# Autodesk Inventor assembly: printer
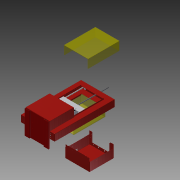
[picture p0: Inventor's stored thumbnail of the model, 180x180]
Saved by Autodesk Inventor 2014 SP2 (Build 180246200, 246)
## iProperties
Created: 2016-09-18
Part Number: printer
Document SubType Name: Assembly
Designer: cruiser
Mass: 5383.42 g
Surface Area: 18310.6 cm^2
Volume: 1570.17 cm^3
Density: 3.42856 g/cm^3
Author: cruiser
## Documents named in this file (18)
- C:\Users\cruiser\Desktop\models\3d printers\laserresin5\printer.iam
- C:\Users\cruiser\Desktop\models\3d printers\laserresin5\frame_front.ipt
- C:\Users\cruiser\Desktop\models\3d printers\laserresin5\frame_back.ipt
- C:\Users\cruiser\Desktop\models\3d printers\laserresin5\drawer.ipt
- C:\Users\cruiser\Desktop\models\3d printers\laserresin5\reservoir.ipt
- C:\Users\cruiser\Desktop\models\3d printers\laserresin5\tray.ipt
- C:\Users\cruiser\Desktop\models\3d printers\laserresin5\crane.ipt
- C:\Users\cruiser\Desktop\models\3d printers\laserresin5\platform.ipt
- C:\Users\cruiser\Desktop\models\3d printers\laserresin5\handle.ipt
- C:\Users\cruiser\Desktop\models\3d printers\laserresin5\laserholder.ipt
- C:\Users\cruiser\Desktop\models\3d printers\laserresin5\nema17.ipt
- C:\Users\cruiser\Desktop\models\3d printers\laserresin5\lmk8luu.ipt
- C:\Users\cruiser\Desktop\models\3d printers\laserresin5\threaded_rod.ipt
- C:\Users\cruiser\Desktop\models\3d printers\laserresin5\shf8.ipt
- C:\Users\cruiser\Desktop\models\3d printers\laserresin5\m8_rail.ipt
- C:\Users\cruiser\Desktop\models\3d printers\laserresin5\foot.ipt
- C:\Users\cruiser\Desktop\models\3d printers\laserresin5\shield.ipt
- C:\Users\cruiser\Desktop\models\3d printers\laserresin5\drawer_pcb.ipt
## Components (24 placed, 17 different names)
1. frame_front:1 — Mate:1, Mate:8, Mate:9, Mate:17, Mate:19, Mate:26, Mate:38, Mate:39, Mate:40, Mate:41, Mate:42, Mate:43, Mate:44, Mate:45, Mate:46, Mate:47, Mate:48, Mate:49, Flush:7, Flush:8, Mate:60, Mate:61, Mate:67
2. frame_back:1 — Mate:60, Mate:61, Mate:64, Mate:65, Mate:66
3. drawer:1 — Mate:1, Mate:19, Mate:23, Mate:24, Mate:26, Mate:54, Mate:57, Mate:58, Mate:59, Mate:62
4. reservoir:1 — Mate:5, Flush:4, Mate:13, Mate:14, Mate:15, Mate:16, Mate:23, Mate:24, Flush:6, Mate:59
5. tray:1 — Mate:5, Flush:4, Flush:6
6. crane:1 — Mate:6, Mate:8, Mate:9, Mate:27, Mate:28, Mate:29, Mate:30, Mate:31, Mate:32, Mate:33, Mate:34, Mate:35, Mate:52, Mate:53
7. platform:1 — Mate:6, Mate:52, Mate:53
8. handle:1 — Mate:13, Mate:14
9. handle:2 — Mate:15, Mate:16
10. laserholder:1 — Mate:17
11. nema17:1 — Mate:27, Mate:28, Mate:29, Mate:36, Mate:37
12. lmk8luu:1 — Mate:30, Mate:34, Mate:35
13. lmk8luu:2 — Mate:31, Mate:32, Mate:33
14. threaded_rod:1 — Mate:36, Mate:37
15. shf8:1 — Mate:44, Mate:45, Mate:46
16. shf8:2 — Mate:41, Mate:42, Mate:43
17. shf8:3 — Mate:47, Mate:48, Mate:49, Mate:51
18. shf8:4 — Mate:38, Mate:39, Mate:40, Mate:50
19. m8_rail:1 — Mate:50, Flush:7
20. m8_rail:2 — Mate:51, Flush:8
21. foot:1 — Mate:54, Mate:57, Mate:58
22. shield:1 — Mate:62
23. shield:2 — Mate:64, Mate:68
24. drawer_pcb:1 — Mate:65, Mate:66, Mate:67, Mate:68
## Relationships (57: Mate 53, Flush 4)
- Mate:1: frame_front:1 ↔ drawer:1
- Mate:5: reservoir:1 ↔ tray:1
- Flush:4: reservoir:1 ↔ tray:1
- Mate:6: crane:1 ↔ platform:1
- Mate:8: frame_front:1 ↔ crane:1
- Mate:9: frame_front:1 ↔ crane:1
- Mate:13: reservoir:1 ↔ handle:1
- Mate:14: reservoir:1 ↔ handle:1
- Mate:15: reservoir:1 ↔ handle:2
- Mate:16: reservoir:1 ↔ handle:2
- Mate:17: frame_front:1 ↔ laserholder:1
- Mate:19: frame_front:1 ↔ drawer:1
- Mate:23: drawer:1 ↔ reservoir:1
- Mate:24: drawer:1 ↔ reservoir:1
- Flush:6: reservoir:1 ↔ tray:1
- Mate:26 (0.1 mm): frame_front:1 ↔ drawer:1
- Mate:27: crane:1 ↔ nema17:1
- Mate:28: crane:1 ↔ nema17:1
- Mate:29: crane:1 ↔ nema17:1
- Mate:30: crane:1 ↔ lmk8luu:1
- Mate:31: crane:1 ↔ lmk8luu:2
- Mate:32: crane:1 ↔ lmk8luu:2
- Mate:33: crane:1 ↔ lmk8luu:2
- Mate:34: crane:1 ↔ lmk8luu:1
- Mate:35: crane:1 ↔ lmk8luu:1
- Mate:36: nema17:1 ↔ threaded_rod:1
- Mate:37: nema17:1 ↔ threaded_rod:1
- Mate:38: frame_front:1 ↔ shf8:4
- Mate:39: frame_front:1 ↔ shf8:4
- Mate:40: frame_front:1 ↔ shf8:4
- Mate:41: frame_front:1 ↔ shf8:2
- Mate:42: frame_front:1 ↔ shf8:2
- Mate:43: frame_front:1 ↔ shf8:2
- Mate:44: frame_front:1 ↔ shf8:1
- Mate:45: frame_front:1 ↔ shf8:1
- Mate:46: frame_front:1 ↔ shf8:1
- Mate:47: frame_front:1 ↔ shf8:3
- Mate:48: frame_front:1 ↔ shf8:3
- Mate:49: frame_front:1 ↔ shf8:3
- Mate:50: shf8:4 ↔ m8_rail:1
- Flush:7: frame_front:1 ↔ m8_rail:1
- Mate:51: shf8:3 ↔ m8_rail:2
- Flush:8: frame_front:1 ↔ m8_rail:2
- Mate:52: crane:1 ↔ platform:1
- Mate:53: crane:1 ↔ platform:1
- Mate:54: drawer:1 ↔ foot:1
- Mate:57: drawer:1 ↔ foot:1
- Mate:58: drawer:1 ↔ foot:1
- Mate:59: drawer:1 ↔ reservoir:1
- Mate:60: frame_front:1 ↔ frame_back:1
- Mate:61: frame_front:1 ↔ frame_back:1
- Mate:62: drawer:1 ↔ shield:1
- Mate:64: frame_back:1 ↔ shield:2
- Mate:65: frame_back:1 ↔ drawer_pcb:1
- Mate:66: frame_back:1 ↔ drawer_pcb:1
- Mate:67: frame_front:1 ↔ drawer_pcb:1
- Mate:68: shield:2 ↔ drawer_pcb:1
